# Autodesk Inventor assembly: DruggerArmAsm
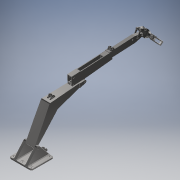
[picture p0: Inventor's stored thumbnail of the model, 180x180]
Saved by Autodesk Inventor 2019 (Build 230136000, 136)
## iProperties
Created: 2018-12-27
Part Number: DruggerArmAsm
Material: 常规
Document SubType Name: Assembly
Designer: JianQiao Hu
Author: JianQiao Hu
## Documents named in this file (8)
- C:\Users\Administrator\Desktop\机械产品数字化设计大赛\月球机器人\机械臂\DruggerArm\DruggerArmAsm.iam
- C:\Users\Administrator\Desktop\机械产品数字化设计大赛\月球机器人\机械臂\DruggerArm\MainArmPed.ipt
- C:\Users\Administrator\Desktop\机械产品数字化设计大赛\月球机器人\机械臂\DruggerArm\MainArm.ipt
- C:\Users\Administrator\Desktop\机械产品数字化设计大赛\月球机器人\机械臂\DruggerArm\DipperParent.ipt
- C:\Users\Administrator\Desktop\机械产品数字化设计大赛\月球机器人\机械臂\DruggerArm\DipperSon.ipt
- C:\Users\Administrator\Desktop\机械产品数字化设计大赛\月球机器人\机械臂\DruggerArm\ConnectBar.ipt
- C:\Users\Administrator\Desktop\机械产品数字化设计大赛\月球机器人\机械臂\DruggerArm\ConnectBoard.ipt
- C:\Users\Administrator\Desktop\机械产品数字化设计大赛\月球机器人\机械臂\DruggerArm\Hand.iam
## Components (8 placed, 7 different names)
1. MainArmPed:1 — 配合:1, 配合:2, 配合:3, 表面齐平:1
2. MainArm:1 — 配合:1, 配合:3, 配合:4, 配合:5
3. DipperParent:1 — 配合:4, 配合:5, 配合:6, 配合:7
4. DipperSon:1 — 配合:6, 配合:7, 配合:10, 配合:11, 配合:13, 配合:15, 表面齐平:2, 配合:20, 配合:21
5. ConnectBar:2 — 配合:10, 配合:11, 配合:17
6. ConnectBar:4 — 配合:13, 配合:15, 配合:18
7. ConnectBoard:1 — 配合:17, 表面齐平:2, 配合:18, 配合:19
8. Hand:1 [sub-assembly] — 配合:19, 配合:20, 配合:21
## Relationships (18: Mate 16, Flush 2)
- 配合:1 [Mate]: MainArmPed:1 ↔ MainArm:1
- 配合:2 [Mate]: MainArmPed:1
- 配合:3 [Mate]: MainArmPed:1 ↔ MainArm:1
- 配合:4 [Mate]: MainArm:1 ↔ DipperParent:1
- 配合:5 [Mate]: MainArm:1 ↔ DipperParent:1
- 表面齐平:1 [Flush]: MainArmPed:1
- 配合:6 [Mate]: DipperParent:1 ↔ DipperSon:1
- 配合:7 [Mate]: DipperParent:1 ↔ DipperSon:1
- 配合:10 [Mate]: DipperSon:1 ↔ ConnectBar:2
- 配合:11 [Mate]: DipperSon:1 ↔ ConnectBar:2
- 配合:13 [Mate]: DipperSon:1 ↔ ConnectBar:4
- 配合:15 [Mate]: DipperSon:1 ↔ ConnectBar:4
- 配合:17 [Mate]: ConnectBar:2 ↔ ConnectBoard:1
- 表面齐平:2 [Flush]: DipperSon:1 ↔ ConnectBoard:1
- 配合:18 [Mate]: ConnectBar:4 ↔ ConnectBoard:1
- 配合:19 [Mate]: ConnectBoard:1 ↔ Hand:1
- 配合:20 [Mate]: DipperSon:1 ↔ Hand:1
- 配合:21 [Mate]: DipperSon:1 ↔ Hand:1
